# Autodesk Inventor assembly: llanta trasera
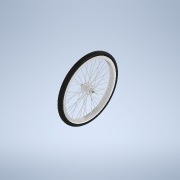
[picture p0: Inventor's stored thumbnail of the model, 180x180]
Saved by Autodesk Inventor 2021 (Build 250183000, 183)
## iProperties
Created: 2021-04-24
Part Number: llanta trasera
Document SubType Name: Assembly
Designer: j2seb
Author: j2seb
## Documents named in this file (6)
- C:\Git\Proyecto_APM\02 Inventor\bicicleta_ruta\otros\llanta trasera.iam
- C:\Git\Proyecto_APM\02 Inventor\bicicleta_ruta\otros\Ensamble_Llanta.iam
- C:\Git\Proyecto_APM\02 Inventor\bicicleta_ruta\otros\eje manzana.ipt
- C:\Git\Proyecto_APM\02 Inventor\bicicleta_playera\Transmision\Design Accelerator\Roller Chain Sprocket11.ipt
- C:\Git\Proyecto_APM\02 Inventor\bicicleta_ruta\otros\retenedor_plato.ipt
- C:\Users\j2seb\OneDrive\Documents\Inventor\Content Center Files\R2021\es-ES\DIN 6923\DIN 6923 - M10 x 1,5.ipt
## Components (8 placed, 5 different names)
1. eje manzana:1 — Coincidencia:6, Coincidencia:9, Coincidencia:11, Mate:12
2. Roller Chain Sprocket1:1 — Coincidencia:4, Mate:16, Mate:17
3. retenedor_plato:1 — Coincidencia:4, Mate:18
4. retenedor_plato:2 — Coincidencia:6, Mate:19, Flush:1
5. Roller Chain Sprocket1:2 — Mate:15, Mate:19
6. DIN 6923 M10:1 — Coincidencia:9
7. DIN 6923 M10:2 — Coincidencia:11
8. Ensamble_Llanta:1 [sub-assembly] — Mate:12, Mate:13, Mate:15, Mate:16, Mate:17, Mate:18, Flush:1
## Relationships (12: Mate 11, Flush 1)
- Coincidencia:4 [Mate]: Roller Chain Sprocket1:1 ↔ retenedor_plato:1
- Coincidencia:6 [Mate]: eje manzana:1 ↔ retenedor_plato:2
- Coincidencia:9 [Mate]: eje manzana:1 ↔ DIN 6923 M10:1
- Coincidencia:11 [Mate]: eje manzana:1 ↔ DIN 6923 M10:2
- Mate:12: eje manzana:1 ↔ Ensamble_Llanta:1
- Mate:13: Ensamble_Llanta:1
- Mate:15: Roller Chain Sprocket1:2 ↔ Ensamble_Llanta:1
- Mate:16: Roller Chain Sprocket1:1 ↔ Ensamble_Llanta:1
- Mate:17: Roller Chain Sprocket1:1 ↔ Ensamble_Llanta:1
- Mate:18: retenedor_plato:1 ↔ Ensamble_Llanta:1
- Mate:19: retenedor_plato:2 ↔ Roller Chain Sprocket1:2
- Flush:1: retenedor_plato:2 ↔ Ensamble_Llanta:1
